# Autodesk Inventor assembly: pcb+led+acy
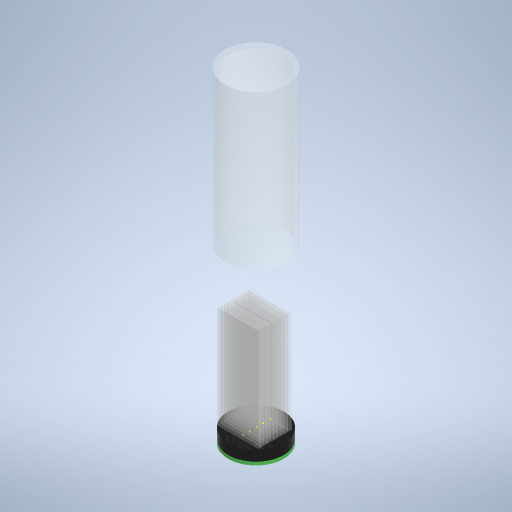
[picture p0: Inventor's stored thumbnail of the model, 512x512]
Saved by Autodesk Inventor 2023 (Build 270158000, 158)
## iProperties
Created: 2022-09-14
Part Number: pcb+led+acy
Document SubType Name: Assembly
Designer: Desmond
Author: Desmond
## Documents named in this file (6)
- G:\LED Nixie Test\Glass Tube\pcb+led+acy.iam
- G:\LED Nixie Test\Glass Tube\Seperator.ipt
- G:\LED Nixie Test\nixie_project.iam
- G:\LED Nixie Test\Glass Tube\Arcylic_Panel_Base_20mm_P1.ipt
- G:\LED Nixie Test\Glass Tube\Arcylic_Panel_Base_20mm_P2.ipt
- G:\LED Nixie Test\Glass Tube\Glass_Tube.ipt
## Components (13 placed, 5 different names)
1. nixie_project:2 [sub-assembly] — Mate:4, Mate:5
2. Seperator:2 — Mate:4, Mate:5, Mate:6, Mate:7, Mate:8, Mate:9, Mate:10, Mate:11, Mate:12, Mate:13, Mate:14, Mate:15, Mate:16, Mate:17, Mate:18, Mate:19, Mate:20, Mate:21, Mate:22, Mate:23, Mate:24, Mate:25, Mate:26, Mate:27, Mate:28, Mate:29, Mate:30, Mate:31, Mate:32, Mate:33, Mate:34, Mate:35, Mate:36
3. Arcylic_Panel_Base_20mm_P1:1 — Mate:11, Mate:21, Mate:30
4. Arcylic_Panel_Base_20mm_P1:2 — Mate:12, Mate:23, Mate:28
5. Arcylic_Panel_Base_20mm_P1:3 — Mate:13, Mate:22, Mate:29
6. Arcylic_Panel_Base_20mm_P1:4 — Mate:14, Mate:25, Mate:26
7. Arcylic_Panel_Base_20mm_P1:5 — Mate:15, Mate:24, Mate:27
8. Arcylic_Panel_Base_20mm_P2:1 — Mate:6, Mate:16, Mate:33
9. Arcylic_Panel_Base_20mm_P2:2 — Mate:7, Mate:17, Mate:32
10. Arcylic_Panel_Base_20mm_P2:3 — Mate:9, Mate:19, Mate:31
11. Arcylic_Panel_Base_20mm_P2:4 — Mate:10, Mate:18, Mate:34
12. Arcylic_Panel_Base_20mm_P2:5 — Mate:8, Mate:20, Mate:35
13. Glass_Tube:1 — Mate:36
## Relationships (33: Mate 33)
- Mate:4: nixie_project:2 ↔ Seperator:2
- Mate:5: nixie_project:2 ↔ Seperator:2
- Mate:6: Seperator:2 ↔ Arcylic_Panel_Base_20mm_P2:1
- Mate:7: Seperator:2 ↔ Arcylic_Panel_Base_20mm_P2:2
- Mate:8: Seperator:2 ↔ Arcylic_Panel_Base_20mm_P2:5
- Mate:9: Seperator:2 ↔ Arcylic_Panel_Base_20mm_P2:3
- Mate:10: Seperator:2 ↔ Arcylic_Panel_Base_20mm_P2:4
- Mate:11: Seperator:2 ↔ Arcylic_Panel_Base_20mm_P1:1
- Mate:12: Seperator:2 ↔ Arcylic_Panel_Base_20mm_P1:2
- Mate:13: Seperator:2 ↔ Arcylic_Panel_Base_20mm_P1:3
- Mate:14: Seperator:2 ↔ Arcylic_Panel_Base_20mm_P1:4
- Mate:15: Seperator:2 ↔ Arcylic_Panel_Base_20mm_P1:5
- Mate:16: Seperator:2 ↔ Arcylic_Panel_Base_20mm_P2:1
- Mate:17: Seperator:2 ↔ Arcylic_Panel_Base_20mm_P2:2
- Mate:18: Seperator:2 ↔ Arcylic_Panel_Base_20mm_P2:4
- Mate:19: Seperator:2 ↔ Arcylic_Panel_Base_20mm_P2:3
- Mate:20: Seperator:2 ↔ Arcylic_Panel_Base_20mm_P2:5
- Mate:21: Seperator:2 ↔ Arcylic_Panel_Base_20mm_P1:1
- Mate:22: Seperator:2 ↔ Arcylic_Panel_Base_20mm_P1:3
- Mate:23: Seperator:2 ↔ Arcylic_Panel_Base_20mm_P1:2
- Mate:24: Seperator:2 ↔ Arcylic_Panel_Base_20mm_P1:5
- Mate:25: Seperator:2 ↔ Arcylic_Panel_Base_20mm_P1:4
- Mate:26: Seperator:2 ↔ Arcylic_Panel_Base_20mm_P1:4
- Mate:27: Seperator:2 ↔ Arcylic_Panel_Base_20mm_P1:5
- Mate:28: Seperator:2 ↔ Arcylic_Panel_Base_20mm_P1:2
- Mate:29: Seperator:2 ↔ Arcylic_Panel_Base_20mm_P1:3
- Mate:30: Seperator:2 ↔ Arcylic_Panel_Base_20mm_P1:1
- Mate:31: Seperator:2 ↔ Arcylic_Panel_Base_20mm_P2:3
- Mate:32: Seperator:2 ↔ Arcylic_Panel_Base_20mm_P2:2
- Mate:33: Seperator:2 ↔ Arcylic_Panel_Base_20mm_P2:1
- Mate:34: Seperator:2 ↔ Arcylic_Panel_Base_20mm_P2:4
- Mate:35: Seperator:2 ↔ Arcylic_Panel_Base_20mm_P2:5
- Mate:36: Seperator:2 ↔ Glass_Tube:1
